# Autodesk Inventor assembly: ChassisDes1
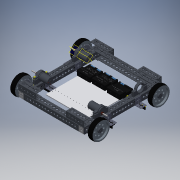
[picture p0: Inventor's stored thumbnail of the model, 180x180]
Saved by Autodesk Inventor 2016 (Build 200138000, 138)
## iProperties
Created: 2015-08-30
Part Number: ChassisDes1
Document SubType Name: Assembly
Designer: Tim
Author: Tim
## Documents named in this file (15)
- C:\Users\Tim\Documents\GitHub\phi_robotics\3d-models\FTC_Tetrix_KOP_Block_Party\Tim Bloot Designs\ChassisDes1.iam
- C:\Users\Tim\Documents\GitHub\phi_robotics\3d-models\FTC_Tetrix_KOP_Block_Party\Tim Bloot Designs\RollingSquareC1.iam
- C:\Users\Tim\Documents\GitHub\phi_robotics\3d-models\FTC_Tetrix_KOP_Block_Party\Tetrix_Kit_FTC\Autodesk Inventor Files\tetrix_corner_bracket.ipt
- C:\Users\Tim\Documents\GitHub\phi_robotics\3d-models\FTC_Tetrix_KOP_Block_Party\Tim Bloot Designs\customLbeam.ipt
- C:\Users\Tim\Documents\GitHub\phi_robotics\3d-models\FTC_Tetrix_KOP_Block_Party\Tetrix_Kit_FTC\Autodesk Inventor Files\tetrix_c_channel-4.ipt
- C:\Users\Tim\Documents\GitHub\phi_robotics\3d-models\FTC_Tetrix_KOP_Block_Party\Tetrix_Kit_FTC\Autodesk Inventor Files\tetrix_c_channel-2.ipt
- C:\Users\Tim\Documents\GitHub\phi_robotics\3d-models\FTC_Tetrix_KOP_Block_Party\Tim Bloot Designs\CustomBasePlate.ipt
- C:\Users\Tim\Documents\GitHub\phi_robotics\3d-models\FTC_Tetrix_KOP_Block_Party\Tetrix_Kit_FTC\Autodesk Inventor Files\tetrix_motor_mount-old.ipt
- C:\Users\Tim\Documents\GitHub\phi_robotics\3d-models\FTC_Tetrix_KOP_Block_Party\Tetrix_Kit_FTC\Autodesk Inventor Files\tetrix_motor.iam
- C:\Users\Tim\Documents\GitHub\phi_robotics\3d-models\FTC_Tetrix_KOP_Block_Party\Tim Bloot Designs\tetrix_motor_screw-long.ipt
- C:\Users\Tim\Documents\GitHub\phi_robotics\3d-models\FTC_Tetrix_KOP_Block_Party\Tetrix_Kit_FTC\Autodesk Inventor Files\tetrix_motor_controller.ipt
- C:\Users\Tim\Documents\GitHub\phi_robotics\3d-models\FTC_Tetrix_KOP_Block_Party\Tetrix_Kit_FTC\Autodesk Inventor Files\tetrix_servo_controller.ipt
- C:\Users\Tim\Documents\GitHub\phi_robotics\3d-models\FTC_Tetrix_KOP_Block_Party\Tetrix_Kit_FTC\Autodesk Inventor Files\tetrix_c_channel-round.ipt
- C:\Users\Tim\Documents\GitHub\phi_robotics\3d-models\FTC_Tetrix_KOP_Block_Party\Tetrix_Kit_FTC\Autodesk Inventor Files\tetrix_screw-short.ipt
- C:\Users\Tim\Documents\GitHub\phi_robotics\3d-models\FTC_Tetrix_KOP_Block_Party\Tetrix_Kit_FTC\Autodesk Inventor Files\tetrix_screw.ipt
## Components (52 placed, 14 different names)
1. tetrix_corner_bracket:1 — Rigid:2, Rigid:33, Rotational:38, Rotational:39
2. tetrix_corner_bracket:2 — Rigid:1, Rotational:42, Rotational:43
3. RollingSquareC1:1 [sub-assembly] — Rigid:1, Rigid:2, Rigid:16, Rigid:17, Rigid:22, Rigid:25, Rigid:27, Rigid:28, Rigid:37, Rigid:38
4. RollingSquareC1:2 [sub-assembly] — Rigid:9, Rigid:10, Rigid:18, Rigid:19, Rigid:23, Rigid:26, Rigid:29, Rotational:32, Rigid:36, Rigid:39
5. tetrix_corner_bracket:7 — Rigid:9, Rigid:32, Rotational:36, Rotational:37
6. tetrix_corner_bracket:8 — Rigid:10, Rotational:48, Rotational:49
7. customLbeam:3 — Rigid:32, Rigid:33
8. customLbeam:4 — Rigid:30, Rigid:31
9. tetrix_corner_bracket:9 — Rigid:16, Rotational:44
10. tetrix_corner_bracket:10 — Rigid:17, Rigid:31, Rotational:40, Rotational:41
11. tetrix_corner_bracket:11 — Rigid:19, Rigid:30, Rotational:34, Rotational:35
12. tetrix_corner_bracket:12 — Rigid:18, Rotational:47
13. tetrix_c_channel-4:1 — Rigid:24
14. tetrix_c_channel-4:2 — Rotational:28
15. tetrix_c_channel-2:1 — Rigid:22, Rigid:24
16. tetrix_c_channel-2:2 — Rigid:23
17. tetrix_c_channel-2:3 — Rigid:25
18. tetrix_c_channel-2:4 — Rigid:26, Rotational:28
19. CustomBasePlate:1
20. tetrix_motor_mount-old:1 — Rigid:27, Rotational:29, Rigid:34, Rigid:35
21. tetrix_motor:1 [sub-assembly] — Rotational:29
22. tetrix_motor_mount-old:2 — Rigid:28, Rotational:30
23. tetrix_motor:2 [sub-assembly] — Rotational:30
24. tetrix_motor_mount-old:3 — Rigid:29, Rotational:31
25. tetrix_motor:3 [sub-assembly] — Rotational:31
26. tetrix_motor_mount-old:4 — Rotational:32, Rotational:33
27. tetrix_motor:4 [sub-assembly] — Rotational:33
28. tetrix_motor_screw-long:1 — Rigid:34
29. tetrix_motor_screw-long:2 — Rigid:35
30. tetrix_motor_controller:2
31. tetrix_motor_controller:3 — Rotational:45
32. tetrix_servo_controller:1 — Rotational:46
33. tetrix_c_channel-round:1 — Rigid:37
34. tetrix_c_channel-round:2 — Rigid:36
35. tetrix_c_channel-round:3 — Rigid:39
36. tetrix_c_channel-round:4 — Rigid:38
37. tetrix_screw-short:1 — Rotational:36
38. tetrix_screw-short:2 — Rotational:37
39. tetrix_screw-short:3 — Rotational:34
40. tetrix_screw-short:4 — Rotational:35
41. tetrix_screw-short:5 — Rotational:43
42. tetrix_screw-short:6 — Rotational:42
43. tetrix_screw-short:7 — Rotational:44
44. tetrix_screw-short:9 — Rotational:48
45. tetrix_screw-short:10 — Rotational:49
46. tetrix_screw-short:11 — Rotational:47
47. tetrix_screw:1 — Rotational:45
48. tetrix_screw:2 — Rotational:46
49. tetrix_screw-short:12 — Rotational:40
50. tetrix_screw-short:13 — Rotational:41
51. tetrix_screw-short:14 — Rotational:38
52. tetrix_screw-short:15 — Rotational:39
## Relationships (48: WeldJoint 26, RevoluteJoint 22)
- Rigid:1 [WeldJoint]: tetrix_corner_bracket:2 ↔ RollingSquareC1:1
- Rigid:2 [WeldJoint]: tetrix_corner_bracket:1 ↔ RollingSquareC1:1
- Rigid:9 [WeldJoint]: RollingSquareC1:2 ↔ tetrix_corner_bracket:7
- Rigid:10 [WeldJoint]: RollingSquareC1:2 ↔ tetrix_corner_bracket:8
- Rigid:16 [WeldJoint]: RollingSquareC1:1 ↔ tetrix_corner_bracket:9
- Rigid:17 [WeldJoint]: RollingSquareC1:1 ↔ tetrix_corner_bracket:10
- Rigid:18 [WeldJoint]: RollingSquareC1:2 ↔ tetrix_corner_bracket:12
- Rigid:19 [WeldJoint]: RollingSquareC1:2 ↔ tetrix_corner_bracket:11
- Rigid:22 [WeldJoint]: RollingSquareC1:1 ↔ tetrix_c_channel-2:1
- Rigid:23 [WeldJoint]: RollingSquareC1:2 ↔ tetrix_c_channel-2:2
- Rigid:24 [WeldJoint]: tetrix_c_channel-4:1 ↔ tetrix_c_channel-2:1
- Rigid:25 [WeldJoint]: RollingSquareC1:1 ↔ tetrix_c_channel-2:3
- Rigid:26 [WeldJoint]: RollingSquareC1:2 ↔ tetrix_c_channel-2:4
- Rotational:28 [RevoluteJoint]: tetrix_c_channel-4:2 ↔ tetrix_c_channel-2:4
- Rigid:27 [WeldJoint]: RollingSquareC1:1 ↔ tetrix_motor_mount-old:1
- Rotational:29 [RevoluteJoint]: tetrix_motor_mount-old:1 ↔ tetrix_motor:1
- Rigid:28 [WeldJoint]: RollingSquareC1:1 ↔ tetrix_motor_mount-old:2
- Rotational:30 [RevoluteJoint]: tetrix_motor_mount-old:2 ↔ tetrix_motor:2
- Rigid:29 [WeldJoint]: RollingSquareC1:2 ↔ tetrix_motor_mount-old:3
- Rotational:31 [RevoluteJoint]: tetrix_motor_mount-old:3 ↔ tetrix_motor:3
- Rotational:32 [RevoluteJoint]: RollingSquareC1:2 ↔ tetrix_motor_mount-old:4
- Rotational:33 [RevoluteJoint]: tetrix_motor_mount-old:4 ↔ tetrix_motor:4
- Rigid:30 [WeldJoint]: customLbeam:4 ↔ tetrix_corner_bracket:11
- Rigid:31 [WeldJoint]: customLbeam:4 ↔ tetrix_corner_bracket:10
- Rigid:32 [WeldJoint]: tetrix_corner_bracket:7 ↔ customLbeam:3
- Rigid:33 [WeldJoint]: tetrix_corner_bracket:1 ↔ customLbeam:3
- Rigid:34 [WeldJoint]: tetrix_motor_mount-old:1 ↔ tetrix_motor_screw-long:1
- Rigid:35 [WeldJoint]: tetrix_motor_mount-old:1 ↔ tetrix_motor_screw-long:2
- Rigid:36 [WeldJoint]: RollingSquareC1:2 ↔ tetrix_c_channel-round:2
- Rigid:37 [WeldJoint]: RollingSquareC1:1 ↔ tetrix_c_channel-round:1
- Rigid:38 [WeldJoint]: RollingSquareC1:1 ↔ tetrix_c_channel-round:4
- Rigid:39 [WeldJoint]: RollingSquareC1:2 ↔ tetrix_c_channel-round:3
- Rotational:34 [RevoluteJoint]: tetrix_corner_bracket:11 ↔ tetrix_screw-short:3
- Rotational:35 [RevoluteJoint]: tetrix_corner_bracket:11 ↔ tetrix_screw-short:4
- Rotational:36 [RevoluteJoint]: tetrix_corner_bracket:7 ↔ tetrix_screw-short:1
- Rotational:37 [RevoluteJoint]: tetrix_corner_bracket:7 ↔ tetrix_screw-short:2
- Rotational:38 [RevoluteJoint]: tetrix_corner_bracket:1 ↔ tetrix_screw-short:14
- Rotational:39 [RevoluteJoint]: tetrix_corner_bracket:1 ↔ tetrix_screw-short:15
- Rotational:40 [RevoluteJoint]: tetrix_corner_bracket:10 ↔ tetrix_screw-short:12
- Rotational:41 [RevoluteJoint]: tetrix_corner_bracket:10 ↔ tetrix_screw-short:13
- Rotational:42 [RevoluteJoint]: tetrix_corner_bracket:2 ↔ tetrix_screw-short:6
- Rotational:43 [RevoluteJoint]: tetrix_corner_bracket:2 ↔ tetrix_screw-short:5
- Rotational:44 [RevoluteJoint]: tetrix_corner_bracket:9 ↔ tetrix_screw-short:7
- Rotational:45 [RevoluteJoint]: tetrix_motor_controller:3 ↔ tetrix_screw:1
- Rotational:46 [RevoluteJoint]: tetrix_servo_controller:1 ↔ tetrix_screw:2
- Rotational:47 [RevoluteJoint]: tetrix_corner_bracket:12 ↔ tetrix_screw-short:11
- Rotational:48 [RevoluteJoint]: tetrix_corner_bracket:8 ↔ tetrix_screw-short:9
- Rotational:49 [RevoluteJoint]: tetrix_corner_bracket:8 ↔ tetrix_screw-short:10
## Named parameters: d9_d4 = 0 mm, d10_d8 = 0 mm
